# Autodesk Inventor assembly: Boba Dispenser 3
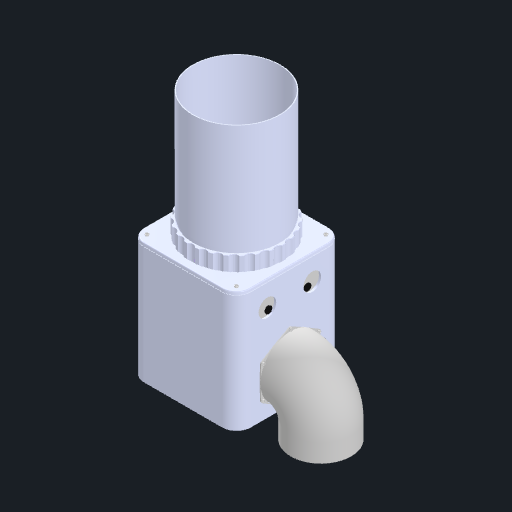
[picture p0: Inventor's stored thumbnail of the model, 512x512]
Saved by Autodesk Inventor 2024 (Build 280153000, 153)
## iProperties
Created: 2024-10-23
Part Number: Boba Dispenser 3
Description: STEP AP214
Document SubType Name: Assembly
Designer: Vincent Larson
Sending System: SolidWorks 2023
Preprocessor: SwSTEP 2.0
Title: assembled  bank.STEP
Author: admin
Revision Number: ANY
## Documents named in this file (20)
- C:\Users\Vincent Larson\Downloads\Boba Dispenser 3.iam
- C:\Users\Vincent Larson\Downloads\assembled  bank\basket adapter.ipt
- C:\Users\Vincent Larson\Downloads\assembled  bank\bottom.ipt
- C:\Users\Vincent Larson\Downloads\assembled  bank\adapter2.ipt
- C:\Users\Vincent Larson\Downloads\assembled  bank\auger.ipt
- C:\Users\Vincent Larson\Downloads\assembled  bank\thread PART.ipt
- C:\Users\Vincent Larson\Downloads\assembled  bank\screw fix holder.ipt
- C:\Users\Vincent Larson\Downloads\assembled  bank\screw_home.ipt
- C:\Users\Vincent Larson\Downloads\assembled  bank\screw holder.ipt
- C:\Users\Vincent Larson\Downloads\assembled  bank\SPHERE_candies.ipt
- C:\Users\Vincent Larson\Downloads\assembled  bank\pan head cross recess screw_iso_ISO 7045 - M2.5 x 8 - Z - 8N.ipt
- C:\Users\Vincent Larson\Downloads\assembled  bank\countersunk flat head cross recess screw_iso_ISO 7046-1 - M3 x 20 - Z - 20N.ipt
- C:\Users\Vincent Larson\Downloads\Boba dispenser 3 bottom.ipt
- C:\Users\Vincent Larson\Downloads\Boba dispenser 3 top.ipt
- C:\Users\Vincent Larson\Downloads\Stepper Motor.ipt
- C:\Users\Vincent Larson\Downloads\Dispenser Tip.ipt
- C:\Users\Vincent Larson\Downloads\Screw\Larson - Screw.ipt
- C:\Users\Vincent Larson\Downloads\Paper piece.ipt
- C:\Users\Vincent Larson\Downloads\eye.ipt
- C:\Users\Vincent Larson\Downloads\Boba Funnel Top 2.ipt
## Components (36 placed, 27 different names)
1. basket adapter_2
2. bottom_3 — Mate:5, Mate:6, Mate:43
3. adapter2_4
4. auger_5 — Mate:17, Mate:18, Mate:19, Flush:1, Mate:21
5. thread PART_7 — Mate:4, Mate:44
6. screw fix holder_9 — Mate:19, Flush:1, Mate:20
7. screw_home_10 — Mate:3
8. screw holder_11 — Mate:17, Mate:18, Mate:20
9. SPHERE_candies_13
10. pan head cross recess screw_iso_ISO 7045 - M2.5 x 8 - Z - 8N_42
11. pan head cross recess screw_iso_ISO 7045 - M2.5 x 8 - Z - 8N_43
12. pan head cross recess screw_iso_ISO 7045 - M2.5 x 8 - Z - 8N_44
13. pan head cross recess screw_iso_ISO 7045 - M2.5 x 8 - Z - 8N_45
14. countersunk flat head cross recess screw_iso_ISO 7046-1 - M3 x 20 - Z - 20N_46
15. countersunk flat head cross recess screw_iso_ISO 7046-1 - M3 x 20 - Z - 20N_47
16. countersunk flat head cross recess screw_iso_ISO 7046-1 - M3 x 20 - Z - 20N_48
17. countersunk flat head cross recess screw_iso_ISO 7046-1 - M3 x 20 - Z - 20N_51 — Mate:2
18. countersunk flat head cross recess screw_iso_ISO 7046-1 - M3 x 20 - Z - 20N_52
19. countersunk flat head cross recess screw_iso_ISO 7046-1 - M3 x 20 - Z - 20N_53
20. Boba dispenser 3 bottom:1 — Mate:2, Mate:3, Mate:24, Mate:25, Mate:26, Mate:27, Mate:28, Mate:29, Mate:35
21. Boba dispenser 3 top:1 — Mate:4, Mate:5, Mate:6, Mate:38, Mate:39, Mate:40, Mate:41, Mate:42
22. Stepper Motor:1 — Mate:21
23. Dispenser Tip:1 — Mate:24, Mate:30, Mate:31, Mate:32, Mate:33, Mate:34, Mate:45, Mate:46
24. Larson - Screw:1 — Mate:26, Mate:32, Mate:45
25. Larson - Screw:2 — Mate:27, Mate:33, Mate:46
26. Larson - Screw:3 — Mate:25, Mate:31
27. Larson - Screw:4 — Mate:29, Mate:30
28. Larson - Screw:5 — Mate:28, Mate:34
29. Paper piece:1 — Mate:35, Mate:36, Mate:37
30. eye:1 — Mate:37
31. eye:2 — Mate:36
32. Larson - Screw:6 — Mate:41, Flush:2
33. Larson - Screw:7 — Mate:38, Flush:4, Mate:42
34. Larson - Screw:8 — Mate:39, Flush:3, Flush:4
35. Larson - Screw:9 — Mate:40, Flush:2, Flush:3
36. Boba Funnel Top 2:1 — Mate:43, Mate:44
## Relationships (37: Mate 33, Flush 4)
- Mate:2: countersunk flat head cross recess screw_iso_ISO 7046-1 - M3 x 20 - Z - 20N_51 ↔ Boba dispenser 3 bottom:1
- Mate:3: screw_home_10 ↔ Boba dispenser 3 bottom:1
- Mate:4: thread PART_7 ↔ Boba dispenser 3 top:1
- Mate:5: bottom_3 ↔ Boba dispenser 3 top:1
- Mate:6: bottom_3 ↔ Boba dispenser 3 top:1
- Mate:17: auger_5 ↔ screw holder_11
- Mate:18: auger_5 ↔ screw holder_11
- Mate:19: auger_5 ↔ screw fix holder_9
- Flush:1: auger_5 ↔ screw fix holder_9
- Mate:20: screw fix holder_9 ↔ screw holder_11
- Mate:21: auger_5 ↔ Stepper Motor:1
- Mate:24: Boba dispenser 3 bottom:1 ↔ Dispenser Tip:1
- Mate:25: Boba dispenser 3 bottom:1 ↔ Larson - Screw:3
- Mate:26: Boba dispenser 3 bottom:1 ↔ Larson - Screw:1
- Mate:27: Boba dispenser 3 bottom:1 ↔ Larson - Screw:2
- Mate:28: Boba dispenser 3 bottom:1 ↔ Larson - Screw:5
- Mate:29: Boba dispenser 3 bottom:1 ↔ Larson - Screw:4
- Mate:30: Dispenser Tip:1 ↔ Larson - Screw:4
- Mate:31: Dispenser Tip:1 ↔ Larson - Screw:3
- Mate:32: Dispenser Tip:1 ↔ Larson - Screw:1
- Mate:33: Dispenser Tip:1 ↔ Larson - Screw:2
- Mate:34: Dispenser Tip:1 ↔ Larson - Screw:5
- Mate:35: Boba dispenser 3 bottom:1 ↔ Paper piece:1
- Mate:36: Paper piece:1 ↔ eye:2
- Mate:37: Paper piece:1 ↔ eye:1
- Mate:38: Boba dispenser 3 top:1 ↔ Larson - Screw:7
- Mate:39: Boba dispenser 3 top:1 ↔ Larson - Screw:8
- Mate:40: Boba dispenser 3 top:1 ↔ Larson - Screw:9
- Mate:41: Boba dispenser 3 top:1 ↔ Larson - Screw:6
- Flush:2: Larson - Screw:6 ↔ Larson - Screw:9
- Flush:3: Larson - Screw:8 ↔ Larson - Screw:9
- Flush:4: Larson - Screw:7 ↔ Larson - Screw:8
- Mate:42: Boba dispenser 3 top:1 ↔ Larson - Screw:7
- Mate:43: bottom_3 ↔ Boba Funnel Top 2:1
- Mate:44: thread PART_7 ↔ Boba Funnel Top 2:1
- Mate:45: Dispenser Tip:1 ↔ Larson - Screw:1
- Mate:46: Dispenser Tip:1 ↔ Larson - Screw:2
